# Autodesk Inventor assembly: Arm1.2ProtoAssembly
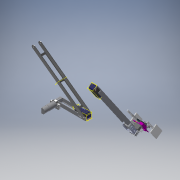
[picture p0: Inventor's stored thumbnail of the model, 180x180]
Saved by Autodesk Inventor 2017 (Build 210142000, 142)
## iProperties
Created: 2017-09-30
Part Number: Arm1.2ProtoAssembly
Document SubType Name: Assembly
Designer: User
Author: User
## Documents named in this file (8)
- C:\Robotics\CAD\2017-18_CAD\ArmProtoAssembly3.0.iam
- C:\Robotics\CAD\2017-18_CAD\ArmProto3.2.ipt
- C:\Robotics\CAD\COTSParts\Tetrix\tetrix-motor-mounts-1.snapshot.1\Tetrex 2pc motor mount.ipt
- C:\Robotics\CAD\COTSParts\Motors\Andymark 2964  NeveRest 40 Motor.ipt
- C:\Robotics\CAD\2017-18_CAD\Claw2017-18.iam
- C:\Robotics\CAD\COTSParts\Motors\REV-41-1300.ipt
- C:\Robotics\CAD\2017-18_CAD\ArmProto2.3.ipt
- C:\Robotics\CAD\2017-18_CAD\ArmProto1.3.ipt
## Components (8 placed, 7 different names)
1. ArmProto3.2:1 — Insert:15, Insert:16, Flush:1, Mate:2
2. Tetrex 2pc motor mount:1 — Insert:9
3. Andymark 2964  NeveRest 40 Motor:1 — Insert:9, Insert:17
4. Claw2017-18:1 [sub-assembly] — Insert:15, Insert:16
5. REV-41-1300:1 — Insert:18, Mate:1, Insert:19, Mate:3
6. ArmProto2.3:1 — Insert:19, Mate:3
7. ArmProto1.3:1 — Insert:17, Insert:18, Mate:1
8. REV-41-1300:2 — Flush:1, Mate:2
## Relationships (10: Insert 6, Mate 3, Flush 1)
- Insert:9: Tetrex 2pc motor mount:1 ↔ Andymark 2964  NeveRest 40 Motor:1
- Insert:15: ArmProto3.2:1 ↔ Claw2017-18:1
- Insert:16: ArmProto3.2:1 ↔ Claw2017-18:1
- Insert:17: Andymark 2964  NeveRest 40 Motor:1 ↔ ArmProto1.3:1
- Insert:18: REV-41-1300:1 ↔ ArmProto1.3:1
- Mate:1 (15.875 mm): REV-41-1300:1 ↔ ArmProto1.3:1
- Insert:19 (4.7625 mm): REV-41-1300:1 ↔ ArmProto2.3:1
- Flush:1: ArmProto3.2:1 ↔ REV-41-1300:2
- Mate:2: ArmProto3.2:1 ↔ REV-41-1300:2
- Mate:3: REV-41-1300:1 ↔ ArmProto2.3:1
